# Autodesk Inventor assembly: Assembly1
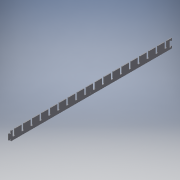
[picture p0: Inventor's stored thumbnail of the model, 180x180]
Saved by Autodesk Inventor 2019 (Build 230136000, 136)
## iProperties
Created: 2019-03-12
Part Number: Assembly1
Document SubType Name: Assembly
Designer: torba
Author: torba
## Documents named in this file (2)
- C:\Users\torba\Nextcloud\Projects\Inventor\Plasma 5x10\Assembly1.iam
- C:\Users\torba\Nextcloud\Projects\Inventor\Plasma 5x10\PLASMA TEMPLATE CUTTING.ipt
## Components (2 placed, 1 different names)
1. PLASMA TEMPLATE CUTTING:1 — Flush:1, Flush:2, Mate:1
2. PLASMA TEMPLATE CUTTING:2 — Flush:1, Flush:2, Mate:1
## Relationships (3: Flush 2, Mate 1)
- Flush:1: PLASMA TEMPLATE CUTTING:1 ↔ PLASMA TEMPLATE CUTTING:2
- Flush:2: PLASMA TEMPLATE CUTTING:1 ↔ PLASMA TEMPLATE CUTTING:2
- Mate:1: PLASMA TEMPLATE CUTTING:1 ↔ PLASMA TEMPLATE CUTTING:2
